# Autodesk Inventor assembly: mech_assembly-left_a
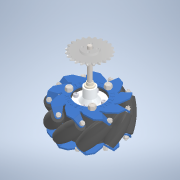
[picture p0: Inventor's stored thumbnail of the model, 180x180]
Saved by Autodesk Inventor 2020 (Build 240168000, 168)
## iProperties
Created: 2019-09-11
Part Number: mech_assembly-left_a
Document SubType Name: Assembly
Designer: tbloo
Author: tbloo
## Documents named in this file (6)
- D:\Documents\GitHub\AO_Robotics\CAD\Projects\Timothy Bloot\mech_assembly-left_a.iam
- D:\Documents\GitHub\AO_Robotics\CAD\Parts Kits\FTC Tetrix KOP Organized (7-24-19)\Wheel\Mechanum Wheel\left_a_mecanum wheel.ipt
- D:\Documents\GitHub\AO_Robotics\CAD\Parts Kits\FTC Tetrix KOP Organized (7-24-19)\Axle Hardware\Tetrix_40225-80mm.ipt
- D:\Documents\GitHub\AO_Robotics\CAD\Parts Kits\FTC Tetrix KOP Organized (7-24-19)\Axle Hardware\AM_6mm_Bushing.ipt
- D:\Documents\GitHub\AO_Robotics\CAD\Parts Kits\FTC Tetrix KOP Organized (7-24-19)\Axle Hardware\Tetrix_39079.iam
- D:\Documents\GitHub\AO_Robotics\CAD\Parts Kits\FTC Tetrix KOP Organized (7-24-19)\Gear\Tetrix_39169.ipt
## Components (6 placed, 5 different names)
1. left_a_mecanum wheel:1 — Rotational:1, Rotational:2
2. Tetrix_40225-80mm:1 — Rotational:2, Rotational:3, Rigid:1
3. AM_6mm_Bushing:1 — Rotational:1
4. AM_6mm_Bushing:2 — Rotational:3
5. Tetrix_39079:1 [sub-assembly] — Rigid:1, Rigid:2
6. Tetrix_39169:1 — Rigid:2
## Relationships (5: RevoluteJoint 3, WeldJoint 2)
- Rotational:1 [RevoluteJoint]: left_a_mecanum wheel:1 ↔ AM_6mm_Bushing:1
- Rotational:2 [RevoluteJoint]: left_a_mecanum wheel:1 ↔ Tetrix_40225-80mm:1
- Rotational:3 [RevoluteJoint] (-18.3 mm): Tetrix_40225-80mm:1 ↔ AM_6mm_Bushing:2
- Rigid:1 [WeldJoint] (-16.3 mm): Tetrix_40225-80mm:1 ↔ Tetrix_39079:1
- Rigid:2 [WeldJoint]: Tetrix_39079:1 ↔ Tetrix_39169:1
